# Autodesk Inventor assembly: Compartment-Assembly-Updated
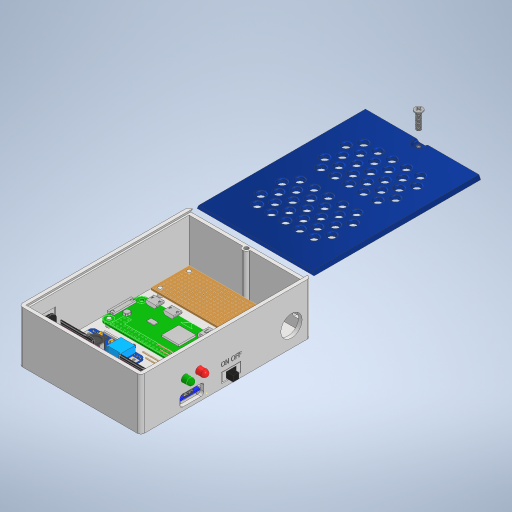
[picture p0: Inventor's stored thumbnail of the model, 512x512]
Saved by Autodesk Inventor 2023 (Build 270158000, 158)
## iProperties
Created: 2024-02-14
Part Number: Compartment-Assembly-Updated
Document SubType Name: Assembly
Designer: ongyu
Author: ongyu
## Documents named in this file (13)
- C:\Users\ongyu\OneDrive\Documents\Inventor\FYP\Electronic-Enclosure\Compartment-Assembly.iam
- C:\Users\ongyu\OneDrive\Documents\Inventor\FYP\Electronic-Enclosure\04-RaspberryPiZeroW.ipt
- C:\Users\ongyu\OneDrive\Documents\Inventor\FYP\Electronic-Enclosure\02-18650-Battery-Holder.ipt
- C:\Users\ongyu\OneDrive\Documents\Inventor\FYP\Electronic-Enclosure\05-TP_4056.ipt
- C:\Users\ongyu\OneDrive\Documents\Inventor\FYP\Electronic-Enclosure\03-MT3608-Module.ipt
- C:\Users\ongyu\OneDrive\Documents\Inventor\FYP\Electronic-Enclosure\07-Green-LED-5mm.ipt
- C:\Users\ongyu\OneDrive\Documents\Inventor\FYP\Electronic-Enclosure\06-Red-LED-5mm.ipt
- C:\Users\ongyu\OneDrive\Documents\Inventor\FYP\Electronic-Enclosure\09-18650-Battery.ipt
- C:\Users\ongyu\OneDrive\Documents\Inventor\FYP\Electronic-Enclosure\11-Small-Switch.ipt
- C:\Users\ongyu\OneDrive\Documents\Inventor\FYP\Electronic-Enclosure\10-Stripboard.ipt
- C:\Users\ongyu\OneDrive\Documents\Inventor\FYP\Electronic-Enclosure\12-Enclosure-Cover.ipt
- C:\Users\ongyu\OneDrive\Documents\Inventor\FYP\Electronic-Enclosure\01-Electronic-Compartment-Height.ipt
- C:\Users\ongyu\OneDrive\Documents\Inventor\FYP\Electronic-Enclosure\13-M3-Screw.ipt
## Components (13 placed, 12 different names)
1. 04-RaspberryPiZeroW:1 — Insert:8, Insert:9
2. 02-18650-Battery-Holder:1 — Insert:5, Mate:6, Mate:7, Mate:8
3. 05-TP_4056:1 — Mate:14
4. 03-MT3608-Module:1 — Mate:11, Mate:12
5. 07-Green-LED-5mm:1 — Insert:11
6. 06-Red-LED-5mm:1 — Insert:10
7. 09-18650-Battery:1 — Insert:5
8. 11-Small-Switch:1 — Mate:2, Mate:3, Flush:2
9. 10-Stripboard:1 — Insert:6, Insert:7
10. 12-Enclosure-Cover:1
11. 01-Electronic-Compartment-Height:1 — Insert:6, Mate:2, Mate:3, Mate:4, Flush:1, Mate:5, Insert:7, Insert:8, Insert:9, Mate:6, Mate:7, Mate:8, Flush:2, Mate:11, Mate:12, Mate:14, Insert:10, Insert:11, Mate:15, Mate:16
12. 12-Enclosure-Cover:2 — Mate:15, Mate:16, Insert:12
13. 13-M3-Screw:1 — Insert:12
## Relationships (22: Mate 12, Insert 8, Flush 2)
- Insert:5: 02-18650-Battery-Holder:1 ↔ 09-18650-Battery:1
- Insert:6: 10-Stripboard:1 ↔ 01-Electronic-Compartment-Height:1
- Mate:2 (0.25 mm): 11-Small-Switch:1 ↔ 01-Electronic-Compartment-Height:1
- Mate:3 (0.25 mm): 11-Small-Switch:1 ↔ 01-Electronic-Compartment-Height:1
- Mate:4: 01-Electronic-Compartment-Height:1
- Flush:1: 01-Electronic-Compartment-Height:1
- Mate:5: 01-Electronic-Compartment-Height:1
- Insert:7: 10-Stripboard:1 ↔ 01-Electronic-Compartment-Height:1
- Insert:8: 04-RaspberryPiZeroW:1 ↔ 01-Electronic-Compartment-Height:1
- Insert:9: 04-RaspberryPiZeroW:1 ↔ 01-Electronic-Compartment-Height:1
- Mate:6: 02-18650-Battery-Holder:1 ↔ 01-Electronic-Compartment-Height:1
- Mate:7: 02-18650-Battery-Holder:1 ↔ 01-Electronic-Compartment-Height:1
- Mate:8: 02-18650-Battery-Holder:1 ↔ 01-Electronic-Compartment-Height:1
- Flush:2: 11-Small-Switch:1 ↔ 01-Electronic-Compartment-Height:1
- Mate:11 (0.05 mm): 03-MT3608-Module:1 ↔ 01-Electronic-Compartment-Height:1
- Mate:12 (1 mm): 03-MT3608-Module:1 ↔ 01-Electronic-Compartment-Height:1
- Mate:14: 05-TP_4056:1 ↔ 01-Electronic-Compartment-Height:1
- Insert:10: 06-Red-LED-5mm:1 ↔ 01-Electronic-Compartment-Height:1
- Insert:11: 07-Green-LED-5mm:1 ↔ 01-Electronic-Compartment-Height:1
- Mate:15: 01-Electronic-Compartment-Height:1 ↔ 12-Enclosure-Cover:2
- Mate:16: 01-Electronic-Compartment-Height:1 ↔ 12-Enclosure-Cover:2
- Insert:12 (10 mm): 12-Enclosure-Cover:2 ↔ 13-M3-Screw:1
